# Autodesk Inventor assembly: KS-15_all
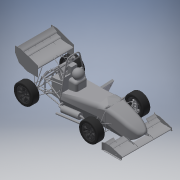
[picture p0: Inventor's stored thumbnail of the model, 180x180]
Saved by Autodesk Inventor 2018 (Build 220112000, 112)
## iProperties
Created: 2018-05-19
Part Number: KS-15_all
Material: 一般
Document SubType Name: Assembly
Designer: ku_sk
Author: ku_sk
## Documents named in this file (15)
- Z:\各班フォルダ\2018\ボディ\エアロ\Aero\KS-15\全体アッセンブリ解析用モデル\KS-15_all.iam
- Z:\各班フォルダ\2018\ボディ\エアロ\Aero\KS-15\全体アッセンブリ解析用モデル\body\parts\2018Frontnose for analysis.ipt
- Z:\各班フォルダ\2018\ボディ\エアロ\Aero\KS-15\全体アッセンブリ解析用モデル\body\parts\SidePanel_Upper for analysis.ipt
- Z:\各班フォルダ\2018\ボディ\エアロ\Aero\KS-15\全体アッセンブリ解析用モデル\body\parts\karikuni12a.ipt
- Z:\各班フォルダ\2018\ボディ\エアロ\Aero\KS-15\全体アッセンブリ解析用モデル\body\intake\2018 Intake.iam
- Z:\各班フォルダ\2018\ボディ\エアロ\Aero\KS-15\全体アッセンブリ解析用モデル\body\engine\simplicity engine.ipt
- Z:\各班フォルダ\2018\ボディ\エアロ\Aero\KS-15\全体アッセンブリ解析用モデル\body\radiator\radiator 2018.ipt
- Z:\各班フォルダ\2018\ボディ\エアロ\Aero\KS-15\全体アッセンブリ解析用モデル\body\exhaust\2018 Exhaust assembly.iam
- Z:\各班フォルダ\2018\ボディ\エアロ\Aero\KS-15\全体アッセンブリ解析用モデル\body\sus\AssyTsutsui2018A.iam
- Z:\各班フォルダ\2018\ボディ\エアロ\Aero\KS-15\全体アッセンブリ解析用モデル\body\sus\F-Upright2018.iam
- Z:\各班フォルダ\2018\ボディ\エアロ\Aero\KS-15\全体アッセンブリ解析用モデル\body\sus\R-Upright2018.iam
- Z:\各班フォルダ\2018\ボディ\エアロ\Aero\KS-15\全体アッセンブリ解析用モデル\body\sus\F-Upright20181.iam
- Z:\各班フォルダ\2018\ボディ\エアロ\Aero\KS-15\全体アッセンブリ解析用モデル\body\sus\R-Upright20181.iam
- Z:\各班フォルダ\2018\ボディ\エアロ\Aero\KS-15\全体アッセンブリ解析用モデル\Rr.wing\simpleRrwing.ipt
- Z:\各班フォルダ\2018\ボディ\エアロ\Aero\KS-15\全体アッセンブリ解析用モデル\Fr.wing\ver.1\newFr.wing_cradle2.ipt
## Components (14 placed, 14 different names)
1. 2018Frontnose for analysis:1 — メイト:5
2. SidePanel_Upper for analysis:1 — フラッシュ:2, メイト:5
3. karikuni12a:1 — メイト:6, メイト:7, メイト:8
4. 2018 Intake:1 [sub-assembly]
5. simplicity engine:1
6. radiator 2018:1
7. 2018 Exhaust assembly:1 [sub-assembly]
8. AssyTsutsui2018A:1 [sub-assembly]
9. F-Upright2018:1 [sub-assembly]
10. R-Upright2018:1 [sub-assembly]
11. F-Upright20181:1 [sub-assembly]
12. R-Upright20181:1 [sub-assembly]
13. simpleRrwing:1
14. newFr.wing_cradle2:1
## Relationships (5: Mate 4, Flush 1)
- フラッシュ:2 [Flush]: SidePanel_Upper for analysis:1
- メイト:5 [Mate]: 2018Frontnose for analysis:1 ↔ SidePanel_Upper for analysis:1
- メイト:6 [Mate]: karikuni12a:1
- メイト:7 [Mate]: karikuni12a:1
- メイト:8 [Mate]: karikuni12a:1
